# Autodesk Inventor assembly: scisor lift 2022
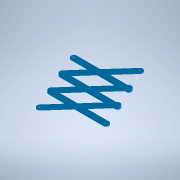
[picture p0: Inventor's stored thumbnail of the model, 180x180]
Saved by Autodesk Inventor 2022 (Build 260153000, 153)
## iProperties
Created: 2023-04-13
Part Number: scisor lift 2022
Document SubType Name: Assembly
Designer: Johnny Jou
Author: Johnny Jou
## Documents named in this file (2)
- C:\Users\Johnny Jou\Documents\GitHub\Areo_Rider_Cabin\Expansion\scisor lift 2022.iam
- C:\Users\Johnny Jou\Documents\GitHub\Areo_Rider_Cabin\Expansion\link_2022.ipt
## Components (6 placed, 1 different names)
1. link_2022:1 — 插入:1, 插入:2
2. link_2022:2 — 插入:1, 插入:3
3. link_2022:3 — 插入:2, 插入:4, 插入:7
4. link_2022:4 — 插入:3, 插入:4, 插入:6
5. link_2022:5 — 插入:6
6. link_2022:6 — 插入:7
## Relationships (7: Insert 7)
- 插入:1 [Insert]: link_2022:1 ↔ link_2022:2
- 插入:2 [Insert]: link_2022:1 ↔ link_2022:3
- 插入:3 [Insert]: link_2022:2 ↔ link_2022:4
- 插入:4 [Insert]: link_2022:3 ↔ link_2022:4
- [Insert]: link_2022:5 ↔ link_2022:6
- 插入:6 [Insert]: link_2022:4 ↔ link_2022:5
- 插入:7 [Insert]: link_2022:3 ↔ link_2022:6
## Named parameters: d4_d3 = 0 mm
